# Autodesk Inventor assembly: axis4
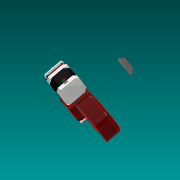
[picture p0: Inventor's stored thumbnail of the model, 180x180]
Saved by Autodesk Inventor 2020.3 (Build 243373000, 373)
## iProperties
Created: 2020-05-24
Part Number: axis4
Document SubType Name: Assembly
Designer: Svend
Author: Svend
## Documents named in this file (18)
- C:\Users\Svend\OneDrive\Documents\GitHub\BeerMinder\3D-model\axis4\axis4.iam
- C:\Users\Svend\OneDrive\Documents\GitHub\BeerMinder\3D-model\pulleys\GT2 Timing Pulley 60T - 8mm as.ipt
- C:\Users\Svend\OneDrive\Documents\GitHub\BeerMinder\3D-model\stepper motors\42BYG Stepper Motor.ipt
- C:\Users\Svend\OneDrive\Documents\GitHub\BeerMinder\3D-model\pulleys\GT2 Pulley 16T - 5mm as.ipt
- C:\Users\Svend\OneDrive\Documents\GitHub\BeerMinder\3D-model\pulleys\Tandriem16naar60T.ipt
- C:\Users\Svend\OneDrive\Documents\GitHub\BeerMinder\3D-model\Base (Axis 1)\asArm2.ipt
- C:\Users\Svend\OneDrive\Documents\GitHub\BeerMinder\3D-model\axis4\asmountAs4.ipt
- C:\Users\Svend\OneDrive\Documents\GitHub\BeerMinder\3D-model\axis4\steppermount.ipt
- C:\Users\Svend\OneDrive\Documents\GitHub\BeerMinder\3D-model\axis4\stepperspacer.ipt
- C:\Users\Svend\OneDrive\Documents\Inventor\Content Center Files\R2020\en-US\ISO 7380-1\ISO 7380-1 - M3 x 10.ipt
- C:\Users\Svend\OneDrive\Documents\Inventor\Content Center Files\R2020\en-US\ISO 4035(2)\ISO 4035 - M3 - ISO.ipt
- C:\Users\Svend\OneDrive\Documents\Inventor\Content Center Files\R2020\en-US\ISO 7380-1\ISO 7380-1 - M3 x 8.ipt
- C:\Users\Svend\OneDrive\Documents\Inventor\Content Center Files\R2020\en-US\ISO 4762(2)\ISO 4762 - M4 x 20ISO.ipt
- C:\Users\Svend\OneDrive\Documents\GitHub\BeerMinder\3D-model\bearings\conische lager.ipt
- C:\Users\Svend\OneDrive\Documents\GitHub\BeerMinder\3D-model\bearings\insertLager.ipt
- C:\Users\Svend\OneDrive\Documents\Inventor\Content Center Files\R2020\en-US\ISO 4762(2)\ISO 4762 - M4 x 40ISO.ipt
- C:\Users\Svend\OneDrive\Documents\Inventor\Content Center Files\R2020\en-US\ISO 4035(2)\ISO 4035 - M4 - ISO.ipt
- C:\Users\Svend\OneDrive\Documents\GitHub\BeerMinder\3D-model\Base (Axis 1)\as4mount v2.ipt
## Components (34 placed, 17 different names)
1. as4mount v2:1 — Mate:9, Mate:10, Flush:1, Flush:2, Angle:2, Flush:8, Mate:17, Mate:18, Mate:31, Mate:32, Mate:33, Mate:34, Mate:35, Mate:36, Mate:37, Insert:5, Insert:6, Insert:7, Insert:8, Insert:9, Insert:10, Insert:11, Insert:12, Insert:13, Mate:39, Flush:9, Mate:43, Mate:38, Mate:46, Mate:48, Flush:52, Flush:53
2. GT2 Timing Pulley 60T - 8mm as:1 — Mate:7, Mate:8, Mate:43, Mate:50, Angle:3
3. 42BYG Stepper Motor:1 — Mate:13, Angle:2, Flush:8, Mate:19, Mate:20, Mate:21, Mate:23, Mate:24, Mate:25, Mate:26
4. GT2 Pulley 16T - 5mm as:1 — Mate:11, Mate:12, Mate:13
5. Tandriem16naar60T:1 — Mate:7, Mate:8, Mate:11, Mate:12
6. asArm2:1 — Mate:49, Mate:50, Mate:51
7. asmountAs4:1 — Mate:9, Mate:10, Flush:1, Flush:2
8. steppermount:1 — Mate:17, Mate:18, Mate:27, Mate:28, Mate:29, Mate:30, Insert:1, Insert:2, Insert:3, Insert:4, Mate:44, Angle:3
9. stepperspacer:1 — Mate:19, Mate:20, Mate:21, Mate:44
10. conische lager:1 — Mate:39, Mate:49, Flush:52, Mate:51
11. insertLager:1 — Flush:9, Flush:53
12. ISO 4762 M4 x 20:1 — Insert:11
13. ISO 4762 M4 x 20:2 — Insert:12
14. ISO 4762 M4 x 20:3 — Insert:13
15. ISO 4762 M4 x 40:1 — Mate:46, Mate:47
16. ISO 4035 M4:1 — Mate:47, Mate:48
17. ISO 7380-1 M3 x 10:1 — Mate:23, Mate:29
18. ISO 7380-1 M3 x 10:2 — Mate:26, Mate:27
19. ISO 7380-1 M3 x 10:3 — Mate:24, Mate:30
20. ISO 7380-1 M3 x 10:4 — Mate:25, Mate:28
21. ISO 4035 M3:1 — Mate:34, Mate:37
22. ISO 4035 M3:2 — Mate:35, Mate:36
23. ISO 4035 M3:3 — Mate:33, Mate:38
24. ISO 4035 M3:4 — Mate:31, Mate:32
25. ISO 7380-1 M3 x 8:1 — Insert:1
26. ISO 7380-1 M3 x 8:2 — Insert:2
27. ISO 7380-1 M3 x 8:3 — Insert:3
28. ISO 7380-1 M3 x 8:4 — Insert:4
29. ISO 4035 M3:5 — Insert:5
30. ISO 4035 M3:6 — Insert:6
31. ISO 4035 M3:7 — Insert:7
32. ISO 4035 M3:8 — Insert:8
33. ISO 4035 M3:9 — Insert:9
34. ISO 4035 M3:10 — Insert:10
## Relationships (58: Mate 37, Insert 13, Flush 6, Angle 2)
- Mate:7: GT2 Timing Pulley 60T - 8mm as:1 ↔ Tandriem16naar60T:1
- Mate:8 (0.5 mm): GT2 Timing Pulley 60T - 8mm as:1 ↔ Tandriem16naar60T:1
- Mate:9: as4mount v2:1 ↔ asmountAs4:1
- Mate:10: as4mount v2:1 ↔ asmountAs4:1
- Flush:1: as4mount v2:1 ↔ asmountAs4:1
- Flush:2: as4mount v2:1 ↔ asmountAs4:1
- Mate:11: GT2 Pulley 16T - 5mm as:1 ↔ Tandriem16naar60T:1
- Mate:12 (0.5 mm): GT2 Pulley 16T - 5mm as:1 ↔ Tandriem16naar60T:1
- Mate:13: 42BYG Stepper Motor:1 ↔ GT2 Pulley 16T - 5mm as:1
- Angle:2 (180 deg): as4mount v2:1 ↔ 42BYG Stepper Motor:1
- Flush:8: as4mount v2:1 ↔ 42BYG Stepper Motor:1
- Mate:17: as4mount v2:1 ↔ steppermount:1
- Mate:18: as4mount v2:1 ↔ steppermount:1
- Mate:19: 42BYG Stepper Motor:1 ↔ stepperspacer:1
- Mate:20: 42BYG Stepper Motor:1 ↔ stepperspacer:1
- Mate:21: 42BYG Stepper Motor:1 ↔ stepperspacer:1
- Mate:23: 42BYG Stepper Motor:1 ↔ ISO 7380-1 M3 x 10:1
- Mate:24: 42BYG Stepper Motor:1 ↔ ISO 7380-1 M3 x 10:3
- Mate:25: 42BYG Stepper Motor:1 ↔ ISO 7380-1 M3 x 10:4
- Mate:26: 42BYG Stepper Motor:1 ↔ ISO 7380-1 M3 x 10:2
- Mate:27: steppermount:1 ↔ ISO 7380-1 M3 x 10:2
- Mate:28: steppermount:1 ↔ ISO 7380-1 M3 x 10:4
- Mate:29: steppermount:1 ↔ ISO 7380-1 M3 x 10:1
- Mate:30: steppermount:1 ↔ ISO 7380-1 M3 x 10:3
- Mate:31: as4mount v2:1 ↔ ISO 4035 M3:4
- Mate:32: as4mount v2:1 ↔ ISO 4035 M3:4
- Mate:33: as4mount v2:1 ↔ ISO 4035 M3:3
- Mate:34: as4mount v2:1 ↔ ISO 4035 M3:1
- Mate:35: as4mount v2:1 ↔ ISO 4035 M3:2
- Mate:36: as4mount v2:1 ↔ ISO 4035 M3:2
- Mate:37: as4mount v2:1 ↔ ISO 4035 M3:1
- Mate:38: as4mount v2:1 ↔ ISO 4035 M3:3
- Insert:1: steppermount:1 ↔ ISO 7380-1 M3 x 8:1
- Insert:2: steppermount:1 ↔ ISO 7380-1 M3 x 8:2
- Insert:3: steppermount:1 ↔ ISO 7380-1 M3 x 8:3
- Insert:4: steppermount:1 ↔ ISO 7380-1 M3 x 8:4
- Insert:5: as4mount v2:1 ↔ ISO 4035 M3:5
- Insert:6: as4mount v2:1 ↔ ISO 4035 M3:6
- Insert:7: as4mount v2:1 ↔ ISO 4035 M3:7
- Insert:8: as4mount v2:1 ↔ ISO 4035 M3:8
- Insert:9: as4mount v2:1 ↔ ISO 4035 M3:9
- Insert:10: as4mount v2:1 ↔ ISO 4035 M3:10
- Insert:11: as4mount v2:1 ↔ ISO 4762 M4 x 20:1
- Insert:12: as4mount v2:1 ↔ ISO 4762 M4 x 20:2
- Insert:13: as4mount v2:1 ↔ ISO 4762 M4 x 20:3
- Mate:39: as4mount v2:1 ↔ conische lager:1
- Flush:9: as4mount v2:1 ↔ insertLager:1
- Mate:43: as4mount v2:1 ↔ GT2 Timing Pulley 60T - 8mm as:1
- Mate:44: steppermount:1 ↔ stepperspacer:1
- Mate:46: as4mount v2:1 ↔ ISO 4762 M4 x 40:1
- Mate:47: ISO 4762 M4 x 40:1 ↔ ISO 4035 M4:1
- Mate:48: as4mount v2:1 ↔ ISO 4035 M4:1
- Mate:49: asArm2:1 ↔ conische lager:1
- Mate:50: GT2 Timing Pulley 60T - 8mm as:1 ↔ asArm2:1
- Angle:3 (0 deg): GT2 Timing Pulley 60T - 8mm as:1 ↔ steppermount:1
- Flush:52: as4mount v2:1 ↔ conische lager:1
- Mate:51 (-11 mm): asArm2:1 ↔ conische lager:1
- Flush:53: as4mount v2:1 ↔ insertLager:1
